# Autodesk Inventor assembly: bondtech_groovemount_extruder-new-fan-2
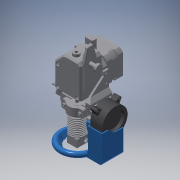
[picture p0: Inventor's stored thumbnail of the model, 180x180]
Saved by Autodesk Inventor 2018 (Build 220112000, 112)
## iProperties
Created: 2019-10-09
Part Number: bondtech_groovemount_extruder-new-fan-2
Description: STEP AP203
Document SubType Name: Assembly
Designer: Vinnie Caprarola
Sending System: SolidWorks 2019
Preprocessor: SwSTEP 2.0
Title: bondtech_groovemount_extruder.STEP
Revision Number: ANY
## Documents named in this file (14)
- Z:\Z\jubilee\cads\tools\direct_drive_bondtech_groovemount_extruder\bondtech_groovemount_extruder-new-fan-2.iam
- Z:\Z\jubilee\cads\tools\direct_drive_bondtech_groovemount_extruder\STEP\groovemount_extruder_base_tool_plate_assembly.iam
- Z:\Z\jubilee\cads\tools\direct_drive_bondtech_groovemount_extruder\STEP\bondtech_bmg_simplified.ipt
- Z:\Z\jubilee\cads\tools\direct_drive_bondtech_groovemount_extruder\STEP\LDO-42STH25-1404MAC.ipt
- Z:\Z\jubilee\cads\tools\direct_drive_bondtech_groovemount_extruder\STEP\m3_6mm_flathead_screw_92125A126_92125A126.ipt
- Z:\Z\jubilee\cads\tools\direct_drive_bondtech_groovemount_extruder\STEP\m3_10mm_buttonhead_screw_92095A182_92095A182.ipt
- Z:\Z\jubilee\cads\tools\direct_drive_bondtech_groovemount_extruder\STEP\m3_40mm_socket_cap_screw_91292A024_91292A024.ipt
- Z:\Z\jubilee\cads\tools\direct_drive_bondtech_groovemount_extruder\STEP\right_parking_wing_assembly.iam
- Z:\Z\jubilee\cads\tools\direct_drive_bondtech_groovemount_extruder\STEP\mounted_extruder_assembly..iam
- Z:\Z\jubilee\cads\tools\direct_drive_bondtech_groovemount_extruder\STEP\m3_6mm_buttonhead_screw_92095A179_92095A179.ipt
- Z:\Z\jubilee\cads\tools\direct_drive_bondtech_groovemount_extruder\STEP\left_parking_wing_assembly.iam
- Z:\Z\jubilee\cads\tools\direct_drive_bondtech_groovemount_extruder\STEP\1.75mm_bowden_tube_adaptor.ipt
- Z:\Z\jubilee\cads\tools\direct_drive_bondtech_groovemount_extruder\FanRing.ipt
- Z:\Z\custom-parts\fan\4020-blower-fan.ipt
## Components (28 placed, 28 different names)
1. groovemount_extruder_base_tool_plate_assembly_1 [sub-assembly] — Flush:9, Flush:10, Flush:12
2. bondtech_bmg_simplified_2
3. LDO-42STH25-1404MAC_3
4. m3_6mm_flathead_screw_92125A126_92125A126_4
5. m3_6mm_flathead_screw_92125A126_92125A126_5
6. m3_6mm_flathead_screw_92125A126_92125A126_6
7. m3_6mm_flathead_screw_92125A126_92125A126_7
8. m3_6mm_flathead_screw_92125A126_92125A126_8
9. m3_6mm_flathead_screw_92125A126_92125A126_9
10. m3_6mm_flathead_screw_92125A126_92125A126_10
11. m3_6mm_flathead_screw_92125A126_92125A126_11
12. m3_10mm_buttonhead_screw_92095A182_92095A182_12
13. m3_10mm_buttonhead_screw_92095A182_92095A182_13
14. m3_10mm_buttonhead_screw_92095A182_92095A182_14
15. m3_10mm_buttonhead_screw_92095A182_92095A182_15
16. m3_40mm_socket_cap_screw_91292A024_91292A024_16
17. m3_40mm_socket_cap_screw_91292A024_91292A024_17
18. m3_40mm_socket_cap_screw_91292A024_91292A024_18
19. right_parking_wing_assembly_19 [sub-assembly] — Mate:1
20. m3_6mm_flathead_screw_92125A126_92125A126_20
21. m3_6mm_flathead_screw_92125A126_92125A126_21
22. mounted_extruder_assembly._22 [sub-assembly] — Flush:2, Flush:3, Flush:4, Flush:5, Flush:11
23. m3_6mm_buttonhead_screw_92095A179_92095A179_23
24. m3_6mm_buttonhead_screw_92095A179_92095A179_24
25. left_parking_wing_assembly_25 [sub-assembly] — Flush:1
26. 1.75mm_bowden_tube_adaptor_26
27. FanRing:1 — Flush:2, Flush:3, Flush:4, Flush:6, Flush:9, Flush:12
28. 4020-blower-fan:1 — Mate:1, Flush:10, Flush:11
## Relationships (11: Flush 10, Mate 1)
- Flush:1 (15 mm): left_parking_wing_assembly_25
- Flush:2: mounted_extruder_assembly._22 ↔ FanRing:1
- Flush:3: mounted_extruder_assembly._22 ↔ FanRing:1
- Flush:4: mounted_extruder_assembly._22 ↔ FanRing:1
- Flush:5 (30 mm): mounted_extruder_assembly._22
- Flush:6: FanRing:1
- Flush:9: groovemount_extruder_base_tool_plate_assembly_1 ↔ FanRing:1
- Mate:1 (3 mm): right_parking_wing_assembly_19 ↔ 4020-blower-fan:1
- Flush:10 (1 mm): groovemount_extruder_base_tool_plate_assembly_1 ↔ 4020-blower-fan:1
- Flush:11 (30 mm): mounted_extruder_assembly._22 ↔ 4020-blower-fan:1
- Flush:12: groovemount_extruder_base_tool_plate_assembly_1 ↔ FanRing:1
